# Autodesk Inventor assembly: Assembly1
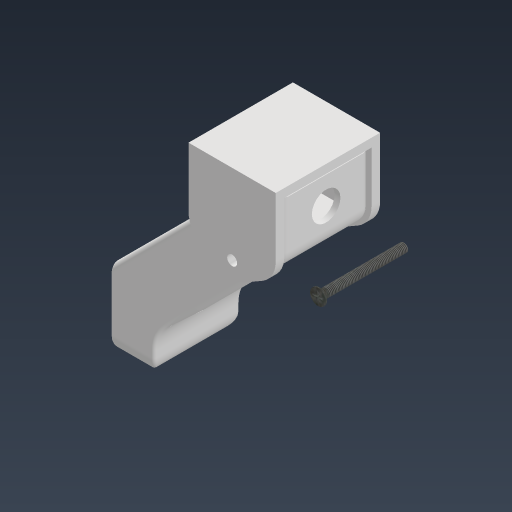
[picture p0: Inventor's stored thumbnail of the model, 512x512]
Saved by Autodesk Inventor 2024 (Build 280153000, 153)
## iProperties
Created: 2023-12-28
Part Number: Assembly1
Document SubType Name: Assembly
Designer: Piter
Author: Piter
## Documents named in this file (4)
- C:\Users\Piter\OneDrive\Pulpit\Modele\My-3D-printing-projects\Filament_cleaner\Assembly1.iam
- C:\Users\Piter\OneDrive\Pulpit\Modele\My-3D-printing-projects\Filament_cleaner\Arm.ipt
- C:\Users\Piter\OneDrive\Pulpit\Modele\My-3D-printing-projects\Filament_cleaner\Cover.ipt
- C:\Users\Piter\OneDrive\Dokumenty\Inventor\Content Center Files\R2024\en-US\ISO 7046-2 H\ISO 7046-2 H - M3x30 - 8.8 - H1.ipt
## Components (3 placed, 3 different names)
1. Arm:1 — Mate:1, Mate:2
2. Cover:2 — Mate:1, Mate:2
3. ISO 7046-2 H M3x30 - 8.8 - H1:1
## Relationships (2: Mate 2)
- Mate:1: Arm:1 ↔ Cover:2
- Mate:2: Arm:1 ↔ Cover:2
